# Autodesk Inventor assembly: V2FullAssembly
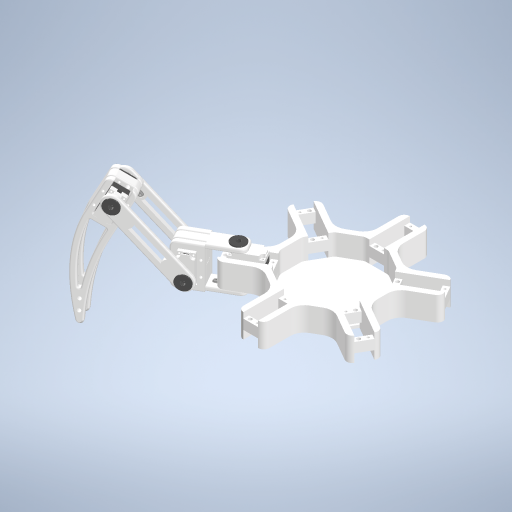
[picture p0: Inventor's stored thumbnail of the model, 512x512]
Saved by Autodesk Inventor 2024 (Build 280153000, 153)
## iProperties
Created: 2026-02-25
Part Number: V2FullAssembly
Document SubType Name: Assembly
Designer: Liam
Author: Liam
## Documents named in this file (3)
- C:\Users\Liam\OneDrive\Documents\Inventor\Hexapod\V2\V2FullAssembly.iam
- C:\Users\Liam\OneDrive\Documents\Inventor\Hexapod\V2\HexBodyBottom.ipt
- C:\Users\Liam\OneDrive\Documents\Inventor\Hexapod\V2\V2Leg.iam
## Components (2 placed, 2 different names)
1. HexBodyBottom:1 — Rigid:1
2. V2Leg:1 [sub-assembly] — Rigid:1
## Relationships (1: WeldJoint 1)
- Rigid:1 [WeldJoint]: HexBodyBottom:1 ↔ V2Leg:1
